# Autodesk Inventor assembly: Assembly_Rymapt_Ethoscope
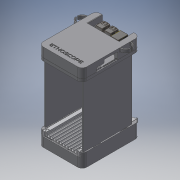
[picture p0: Inventor's stored thumbnail of the model, 180x180]
Saved by Autodesk Inventor 2017 (Build 210142000, 142)
## iProperties
Created: 2017-05-29
Part Number: Assembly_Rymapt_Ethoscope
Document SubType Name: Assembly
Designer: Paolo
Author: Paolo
## Documents named in this file (13)
- E:\Rymapt_projects\Ethoscope\ethoscope_hardware\core_Rymapt\Assembly_Rymapt_Ethoscope.iam
- E:\Rymapt_projects\Ethoscope\ethoscope_hardware\core_Rymapt\LightBox\core_lightBox_new.ipt
- E:\Rymapt_projects\Ethoscope\ethoscope_hardware\arenas\arena_10x1_longTubes\arena_10x1_longTubes.ipt
- E:\Rymapt_projects\Ethoscope\ethoscope_hardware\core\RPi3\RPi3_ModelB.ipt
- E:\Rymapt_projects\Ethoscope\ethoscope_hardware\core_Rymapt\PiCase\upperPiCase_R.ipt
- E:\Rymapt_projects\Ethoscope\ethoscope_hardware\core_Rymapt\PiCase\lowerPiCase_R.ipt
- E:\Rymapt_projects\Ethoscope\ethoscope_hardware\extra\Screws\M2_phillip_8mm.ipt
- E:\Rymapt_projects\Ethoscope\ethoscope_hardware\core\RPi3\RasPi_Camera.ipt
- E:\Rymapt_projects\Ethoscope\ethoscope_hardware\extra\Screws\M2_nut.ipt
- E:\Rymapt_projects\Ethoscope\ethoscope_hardware\extra\Screws\M3_philips_6mm.ipt
- E:\Rymapt_projects\Ethoscope\ethoscope_hardware\core_Rymapt\LightBox\core_lightStrip_R.ipt
- E:\Rymapt_projects\Ethoscope\ethoscope_hardware\extra\Screws\M3_hex_12mm.ipt
- E:\Rymapt_projects\Ethoscope\ethoscope_hardware\core_Rymapt\LightBox\sideWall_r.ipt
## Components (19 placed, 13 different names)
1. sideWall_R:1 — Mate:59, Mate:60, Mate:61, Mate:62
2. sideWall_R:2 — Mate:63, Mate:64, Mate:65
3. M2_nut:2 — Mate:36, Mate:37
4. M2_nut:1 — Mate:34, Mate:35
5. Camera_PiNoir:1 — Mate:14, Mate:32, Mate:33, Mate:34, Mate:36
6. M2_phillip_8mm:2 — Mate:30, Mate:31, Mate:33, Mate:37
7. M2_phillip_8mm:1 — Mate:16, Mate:29, Mate:32, Mate:35
8. M2.5_philips_6mm:1 — Mate:39, Mate:40, Mate:41
9. M3_philips_6mm:2 — Mate:42, Mate:43, Mate:44
10. RPi3_ModelB:1 — Mate:38, Mate:39, Mate:41, Mate:42, Mate:44
11. M2.5_hex_12mm:1 — Mate:50, Mate:57
12. M2.5_hex_12mm:2 — Mate:52, Mate:55
13. M2.5_hex_12mm:3 — Mate:48, Mate:54, Mate:56
14. M2.5_hex_12mm:4 — Mate:46, Mate:53, Mate:58
15. lowerPiCase_R:1 — Flush:1, Flush:2, Pi_Upper_Lower_Z, Mate:14, Mate:16, Mate:29, Mate:30, Mate:31, Mate:38, Mate:40, Mate:43, Mate:53, Mate:54, Mate:55, Mate:56, Mate:57, Mate:58, Mate:59, Mate:62, Mate:64
16. upperPiCase_R:1 — Pi_Upper_Lower_Z, Mate:46, Mate:48, Mate:50, Mate:52
17. arena_10x1_longTubes:1 — Mate:1, Mate:2, Mate:3
18. core_lightBox_new:1 — Mate:1, Mate:2, Mate:3, Flush:1, Flush:2, Mate:25, Mate:26, Mate:27, Mate:60, Mate:61, Mate:63, Mate:65
19. core_lightStrip_R:1 — Mate:25, Mate:26, Mate:27
## Relationships (44: Mate 42, Flush 2)
- Mate:1: arena_10x1_longTubes:1 ↔ core_lightBox_new:1
- Mate:2: arena_10x1_longTubes:1 ↔ core_lightBox_new:1
- Mate:3: arena_10x1_longTubes:1 ↔ core_lightBox_new:1
- Flush:1: lowerPiCase_R:1 ↔ core_lightBox_new:1
- Flush:2: lowerPiCase_R:1 ↔ core_lightBox_new:1
- Pi_Upper_Lower_Z [Mate] (0.2 mm): lowerPiCase_R:1 ↔ upperPiCase_R:1
- Mate:14 (0.2 mm): Camera_PiNoir:1 ↔ lowerPiCase_R:1
- Mate:16 (0.1 mm): M2_phillip_8mm:1 ↔ lowerPiCase_R:1
- Mate:25 (0.1 mm): core_lightBox_new:1 ↔ core_lightStrip_R:1
- Mate:26 (0.1 mm): core_lightBox_new:1 ↔ core_lightStrip_R:1
- Mate:27 (0.2 mm): core_lightBox_new:1 ↔ core_lightStrip_R:1
- Mate:29: M2_phillip_8mm:1 ↔ lowerPiCase_R:1
- Mate:30 (0.1 mm): M2_phillip_8mm:2 ↔ lowerPiCase_R:1
- Mate:31: M2_phillip_8mm:2 ↔ lowerPiCase_R:1
- Mate:32: Camera_PiNoir:1 ↔ M2_phillip_8mm:1
- Mate:33: Camera_PiNoir:1 ↔ M2_phillip_8mm:2
- Mate:34 (0.2 mm): M2_nut:1 ↔ Camera_PiNoir:1
- Mate:35: M2_nut:1 ↔ M2_phillip_8mm:1
- Mate:36: M2_nut:2 ↔ Camera_PiNoir:1
- Mate:37: M2_nut:2 ↔ M2_phillip_8mm:2
- Mate:38 (0.1 mm): RPi3_ModelB:1 ↔ lowerPiCase_R:1
- Mate:39: M2.5_philips_6mm:1 ↔ RPi3_ModelB:1
- Mate:40: M2.5_philips_6mm:1 ↔ lowerPiCase_R:1
- Mate:41 (0.1 mm): M2.5_philips_6mm:1 ↔ RPi3_ModelB:1
- Mate:42: M3_philips_6mm:2 ↔ RPi3_ModelB:1
- Mate:43: M3_philips_6mm:2 ↔ lowerPiCase_R:1
- Mate:44 (0.1 mm): M3_philips_6mm:2 ↔ RPi3_ModelB:1
- Mate:46: M2.5_hex_12mm:4 ↔ upperPiCase_R:1
- Mate:48: M2.5_hex_12mm:3 ↔ upperPiCase_R:1
- Mate:50: M2.5_hex_12mm:1 ↔ upperPiCase_R:1
- Mate:52: M2.5_hex_12mm:2 ↔ upperPiCase_R:1
- Mate:53: M2.5_hex_12mm:4 ↔ lowerPiCase_R:1
- Mate:54: M2.5_hex_12mm:3 ↔ lowerPiCase_R:1
- Mate:55 (0.2 mm): M2.5_hex_12mm:2 ↔ lowerPiCase_R:1
- Mate:56 (0.2 mm): M2.5_hex_12mm:3 ↔ lowerPiCase_R:1
- Mate:57 (0.2 mm): M2.5_hex_12mm:1 ↔ lowerPiCase_R:1
- Mate:58 (0.2 mm): M2.5_hex_12mm:4 ↔ lowerPiCase_R:1
- Mate:59 (0.2 mm): sideWall_R:1 ↔ lowerPiCase_R:1
- Mate:60 (0.2 mm): sideWall_R:1 ↔ core_lightBox_new:1
- Mate:61 (0.1 mm): sideWall_R:1 ↔ core_lightBox_new:1
- Mate:62 (0.1 mm): sideWall_R:1 ↔ lowerPiCase_R:1
- Mate:63 (0.2 mm): sideWall_R:2 ↔ core_lightBox_new:1
- Mate:64 (0.1 mm): sideWall_R:2 ↔ lowerPiCase_R:1
- Mate:65 (0.1 mm): sideWall_R:2 ↔ core_lightBox_new:1
